# Autodesk Inventor assembly: SwalllowMountAssembly
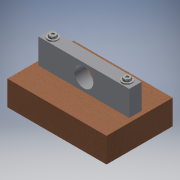
[picture p0: Inventor's stored thumbnail of the model, 180x180]
Saved by Autodesk Inventor 2019.4 (Build 234330000, 330)
## iProperties
Created: 2019-04-05
Part Number: SwalllowMountAssembly
Document SubType Name: Assembly
Designer: steele
Author: steele
## Documents named in this file (4)
- C:\git\CAD-Development\robSteele\HouseProjects\SwallowMount\SwalllowMountAssembly.iam
- C:\git\CAD-Development\robSteele\HouseProjects\BaseOfSwallowWaterer.ipt
- C:\git\CAD-Development\robSteele\HouseProjects\SwallowMount\WoodHandRail.ipt
- C:\git\CAD-Development\robSteele\HouseProjects\SwallowMount\SwalllowMountAssembly\Design Accelerator\Bolted Connection1.iam
## Components (4 placed, 3 different names)
1. BaseOfSwallowWaterer:1 — Mate:1, Flush:1, Flush:2, Mate:2, Flush:4
2. BaseOfSwallowWaterer:2 — Mate:1, Flush:1, Flush:2, Flush:3, Mate:3, Mate:4
3. WoodHandRail:1 — Flush:3, Mate:2, Flush:4
4. Bolted Connection:1 [sub-assembly] — Mate:3, Mate:4
## Relationships (8: Mate 4, Flush 4)
- Mate:1: BaseOfSwallowWaterer:1 ↔ BaseOfSwallowWaterer:2
- Flush:1: BaseOfSwallowWaterer:1 ↔ BaseOfSwallowWaterer:2
- Flush:2: BaseOfSwallowWaterer:1 ↔ BaseOfSwallowWaterer:2
- Flush:3: BaseOfSwallowWaterer:2 ↔ WoodHandRail:1
- Mate:2: BaseOfSwallowWaterer:1 ↔ WoodHandRail:1
- Flush:4: BaseOfSwallowWaterer:1 ↔ WoodHandRail:1
- Mate:3: BaseOfSwallowWaterer:2 ↔ Bolted Connection:1
- Mate:4: BaseOfSwallowWaterer:2 ↔ Bolted Connection:1
